# Autodesk Inventor assembly: emsamble caja
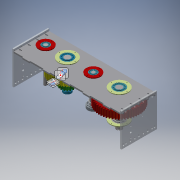
[picture p0: Inventor's stored thumbnail of the model, 180x180]
Saved by Autodesk Inventor 2016 (Build 200138000, 138)
## iProperties
Created: 2017-08-31
Part Number: emsamble caja
Material: Genérico
Document SubType Name: Assembly
Designer: Alumno
Author: Alumno
## Documents named in this file (20)
- C:\Users\Alumno\Desktop\proyecto caja reductora\emsamble caja.iam
- C:\Users\Alumno\Desktop\proyecto caja reductora\Acople N°1.ipt
- C:\Users\Alumno\Desktop\proyecto caja reductora\Plano 2.ipt
- C:\Users\Alumno\Desktop\proyecto caja reductora\AcoplecN°2.ipt
- C:\Users\Alumno\Desktop\proyecto caja reductora\EJE 2 (30 mm y 15 mm).iam
- C:\Users\Alumno\Desktop\proyecto caja reductora\TREN 1\Design Accelerator\Engranaje recto12.ipt
- C:\Users\Alumno\Desktop\proyecto caja reductora\TREN 1\Design Accelerator\Engranaje recto22.ipt
- C:\Users\Alumno\Desktop\proyecto caja reductora\TREN 2\Design Accelerator\Engranaje recto11.ipt
- C:\Users\Alumno\Desktop\proyecto caja reductora\TREN 2\Design Accelerator\Engranaje recto21.ipt
- C:\Users\Alumno\Desktop\proyecto caja reductora\TREN 3\Design Accelerator\Engranaje recto11.ipt
- C:\Users\Alumno\Desktop\proyecto caja reductora\TREN 3\Design Accelerator\Engranaje recto21.ipt
- C:\Users\Alumno\Desktop\proyecto caja reductora\EJE 3 (30-45).iam
- C:\Users\Alumno\Desktop\proyecto caja reductora\EJE 4.iam
- C:\Users\Alumno\Desktop\proyecto caja reductora\Chaveta- Tren 1.ipt
- C:\Users\Alumno\Desktop\proyecto caja reductora\Chaveta 25.ipt
- C:\Users\Alumno\Desktop\proyecto caja reductora\EJE 1.iam
- C:\Users\Alumno\Desktop\proyecto caja reductora\RODAMIENTO 15 D\6002.iam
- C:\Users\Alumno\Desktop\proyecto caja reductora\RODAMIENTO 25 D\6005.iam
- C:\Users\Alumno\Desktop\proyecto caja reductora\PLANO  N°1.ipt
- C:\Users\Alumno\Desktop\proyecto caja reductora\PLANO N°2.ipt
## Components (33 placed, 15 different names)
1. Engranaje recto1:1 — Rotación:4, Coincidencia:138, Coincidencia:139, Coincidencia:184
2. Engranaje recto2:1 — Coincidencia:120, Coincidencia:121, Coincidencia:132, Rotación:4
3. Engranaje recto2:2 — Coincidencia:212, Coincidencia:213, Coincidencia:214, Rotación:7
4. Engranaje recto1:3 — Coincidencia:99, Coincidencia:114, Coincidencia:135, Rotación:6
5. Engranaje recto2:3 — Coincidencia:112, Coincidencia:125, Rotación:6, Coincidencia:206
6. EJE 2 (30 mm y 15 mm):3 [sub-assembly] — Coincidencia:94, Coincidencia:95, Coincidencia:117, Coincidencia:118, Coincidencia:119, Coincidencia:120, Coincidencia:132, Coincidencia:134, Coincidencia:202, Nivelación:5, Coincidencia:230
7. Engranaje recto1:4 — Coincidencia:94, Coincidencia:95, Coincidencia:134, Rotación:7
8. EJE 3 (30-45):1 [sub-assembly] — Coincidencia:99, Coincidencia:114, Coincidencia:127, Coincidencia:128, Coincidencia:129, Coincidencia:135, Coincidencia:203, Nivelación:6, Coincidencia:205, Coincidencia:213, Coincidencia:214
9. EJE 4:1 [sub-assembly] — Coincidencia:112, Coincidencia:122, Coincidencia:123, Coincidencia:124, Coincidencia:204, Nivelación:7, Coincidencia:206
10. Chaveta- Tren 1:1 — Coincidencia:117, Coincidencia:118, Coincidencia:119, Coincidencia:121
11. Chaveta- Tren 1:2 — Coincidencia:122, Coincidencia:123, Coincidencia:124, Coincidencia:125
12. Chaveta 25:6 — Coincidencia:127, Coincidencia:128, Coincidencia:129, Coincidencia:205, Coincidencia:212
13. EJE 1:1 [sub-assembly] — Coincidencia:138, Coincidencia:139, Coincidencia:169, Coincidencia:184, Coincidencia:201, Nivelación:4, Coincidencia:229
14. 6002:3 [sub-assembly] — Coincidencia:169, Coincidencia:197, Nivelación:1, Coincidencia:201, Nivelación:4
15. 6002:4 [sub-assembly] — Coincidencia:199, Nivelación:2, Coincidencia:203, Nivelación:6
16. 6005:3 [sub-assembly] — Coincidencia:200, Nivelación:3, Coincidencia:204, Nivelación:7
17. PLANO  N°1:1 — Coincidencia:185, Coincidencia:186, Coincidencia:187, Coincidencia:188, Coincidencia:189, Coincidencia:190, Coincidencia:191, Coincidencia:192, Coincidencia:193, Coincidencia:194, Coincidencia:195, Coincidencia:196, Nivelación:9, Coincidencia:208, Coincidencia:209, Coincidencia:233, Nivelación:15, Coincidencia:234
18. Acople N°1:2 — Coincidencia:186, Coincidencia:188, Coincidencia:189, Coincidencia:197, Nivelación:1
19. Acople N°1:3 — Coincidencia:185, Coincidencia:187, Coincidencia:190, Coincidencia:199, Nivelación:2
20. AcoplecN°2:1 — Coincidencia:191, Coincidencia:194, Coincidencia:196, Coincidencia:198, Nivelación:8
21. AcoplecN°2:2 — Coincidencia:192, Coincidencia:193, Coincidencia:195, Coincidencia:200, Nivelación:3
22. 6005:5 [sub-assembly] — Coincidencia:198, Coincidencia:202, Nivelación:5, Nivelación:8
23. Plano 2:1 — Nivelación:9, Coincidencia:208, Coincidencia:209, Nivelación:10, Coincidencia:215, Coincidencia:216
24. PLANO N°2:1 — Nivelación:10, Coincidencia:215, Coincidencia:216, Coincidencia:217, Coincidencia:218, Coincidencia:219, Coincidencia:220, Coincidencia:221, Coincidencia:222, Coincidencia:223, Coincidencia:224, Coincidencia:225, Coincidencia:226, Coincidencia:227, Coincidencia:228
25. AcoplecN°2:3 — Coincidencia:218, Coincidencia:222, Coincidencia:226, Coincidencia:231, Nivelación:13
26. Acople N°1:4 — Coincidencia:219, Coincidencia:223, Coincidencia:228, Nivelación:12
27. AcoplecN°2:4 — Coincidencia:217, Coincidencia:221, Coincidencia:227, Coincidencia:232, Nivelación:14
28. Acople N°1:5 — Coincidencia:220, Coincidencia:224, Coincidencia:225, Nivelación:11
29. 6002:5 [sub-assembly] — Coincidencia:229, Nivelación:11
30. 6002:6 [sub-assembly] — Coincidencia:230, Nivelación:12
31. 6005:6 [sub-assembly] — Coincidencia:231, Nivelación:13
32. 6005:7 [sub-assembly] — Coincidencia:232, Nivelación:14
33. Plano 2:2 — Coincidencia:233, Nivelación:15, Coincidencia:234
## Relationships (89: Mate 71, Flush 15, RelateRotation 3)
- Coincidencia:94 [Mate]: EJE 2 (30 mm y 15 mm):3 ↔ Engranaje recto1:4
- Coincidencia:95 [Mate]: EJE 2 (30 mm y 15 mm):3 ↔ Engranaje recto1:4
- Coincidencia:99 [Mate]: Engranaje recto1:3 ↔ EJE 3 (30-45):1
- Coincidencia:112 [Mate]: Engranaje recto2:3 ↔ EJE 4:1
- Coincidencia:114 [Mate]: Engranaje recto1:3 ↔ EJE 3 (30-45):1
- Coincidencia:117 [Mate]: EJE 2 (30 mm y 15 mm):3 ↔ Chaveta- Tren 1:1
- Coincidencia:118 [Mate]: EJE 2 (30 mm y 15 mm):3 ↔ Chaveta- Tren 1:1
- Coincidencia:119 [Mate]: EJE 2 (30 mm y 15 mm):3 ↔ Chaveta- Tren 1:1
- Coincidencia:120 [Mate]: Engranaje recto2:1 ↔ EJE 2 (30 mm y 15 mm):3
- Coincidencia:121 [Mate]: Engranaje recto2:1 ↔ Chaveta- Tren 1:1
- Coincidencia:122 [Mate]: EJE 4:1 ↔ Chaveta- Tren 1:2
- Coincidencia:123 [Mate]: EJE 4:1 ↔ Chaveta- Tren 1:2
- Coincidencia:124 [Mate]: EJE 4:1 ↔ Chaveta- Tren 1:2
- Coincidencia:125 [Mate]: Engranaje recto2:3 ↔ Chaveta- Tren 1:2
- Coincidencia:127 [Mate]: EJE 3 (30-45):1 ↔ Chaveta 25:6
- Coincidencia:128 [Mate]: EJE 3 (30-45):1 ↔ Chaveta 25:6
- Coincidencia:129 [Mate]: EJE 3 (30-45):1 ↔ Chaveta 25:6
- Coincidencia:132 [Mate]: Engranaje recto2:1 ↔ EJE 2 (30 mm y 15 mm):3
- Coincidencia:134 [Mate]: EJE 2 (30 mm y 15 mm):3 ↔ Engranaje recto1:4
- Coincidencia:135 [Mate]: Engranaje recto1:3 ↔ EJE 3 (30-45):1
- Rotación:4 [RelateRotation] (0.3333 ul): Engranaje recto1:1 ↔ Engranaje recto2:1
- Rotación:6 [RelateRotation] (0.3333 ul): Engranaje recto1:3 ↔ Engranaje recto2:3
- Coincidencia:138 [Mate]: Engranaje recto1:1 ↔ EJE 1:1
- Coincidencia:139 [Mate]: Engranaje recto1:1 ↔ EJE 1:1
- Coincidencia:169 [Mate]: EJE 1:1 ↔ 6002:3
- Coincidencia:184 [Mate]: Engranaje recto1:1 ↔ EJE 1:1
- Coincidencia:185 [Mate]: PLANO  N°1:1 ↔ Acople N°1:3
- Coincidencia:186 [Mate]: PLANO  N°1:1 ↔ Acople N°1:2
- Coincidencia:187 [Mate]: PLANO  N°1:1 ↔ Acople N°1:3
- Coincidencia:188 [Mate]: PLANO  N°1:1 ↔ Acople N°1:2
- Coincidencia:189 [Mate]: PLANO  N°1:1 ↔ Acople N°1:2
- Coincidencia:190 [Mate]: PLANO  N°1:1 ↔ Acople N°1:3
- Coincidencia:191 [Mate]: PLANO  N°1:1 ↔ AcoplecN°2:1
- Coincidencia:192 [Mate]: PLANO  N°1:1 ↔ AcoplecN°2:2
- Coincidencia:193 [Mate]: PLANO  N°1:1 ↔ AcoplecN°2:2
- Coincidencia:194 [Mate]: PLANO  N°1:1 ↔ AcoplecN°2:1
- Coincidencia:195 [Mate]: PLANO  N°1:1 ↔ AcoplecN°2:2
- Coincidencia:196 [Mate]: PLANO  N°1:1 ↔ AcoplecN°2:1
- Coincidencia:197 [Mate]: 6002:3 ↔ Acople N°1:2
- Nivelación:1 [Flush]: 6002:3 ↔ Acople N°1:2
- Coincidencia:198 [Mate]: AcoplecN°2:1 ↔ 6005:5
- Coincidencia:199 [Mate]: 6002:4 ↔ Acople N°1:3
- Nivelación:2 [Flush]: 6002:4 ↔ Acople N°1:3
- Coincidencia:200 [Mate]: 6005:3 ↔ AcoplecN°2:2
- Nivelación:3 [Flush]: 6005:3 ↔ AcoplecN°2:2
- Coincidencia:201 [Mate]: EJE 1:1 ↔ 6002:3
- Nivelación:4 [Flush]: EJE 1:1 ↔ 6002:3
- Coincidencia:202 [Mate]: EJE 2 (30 mm y 15 mm):3 ↔ 6005:5
- Nivelación:5 [Flush]: EJE 2 (30 mm y 15 mm):3 ↔ 6005:5
- Coincidencia:203 [Mate]: EJE 3 (30-45):1 ↔ 6002:4
- Nivelación:6 [Flush]: EJE 3 (30-45):1 ↔ 6002:4
- Coincidencia:204 [Mate]: EJE 4:1 ↔ 6005:3
- Nivelación:7 [Flush]: EJE 4:1 ↔ 6005:3
- Coincidencia:205 [Mate]: EJE 3 (30-45):1 ↔ Chaveta 25:6
- Coincidencia:206 [Mate]: Engranaje recto2:3 ↔ EJE 4:1
- Nivelación:8 [Flush]: AcoplecN°2:1 ↔ 6005:5
- Nivelación:9 [Flush]: PLANO  N°1:1 ↔ Plano 2:1
- Coincidencia:208 [Mate]: PLANO  N°1:1 ↔ Plano 2:1
- Coincidencia:209 [Mate]: PLANO  N°1:1 ↔ Plano 2:1
- Coincidencia:212 [Mate]: Engranaje recto2:2 ↔ Chaveta 25:6
- Coincidencia:213 [Mate]: Engranaje recto2:2 ↔ EJE 3 (30-45):1
- Coincidencia:214 [Mate]: Engranaje recto2:2 ↔ EJE 3 (30-45):1
- Rotación:7 [RelateRotation] (0.3333 ul): Engranaje recto2:2 ↔ Engranaje recto1:4
- Nivelación:10 [Flush]: Plano 2:1 ↔ PLANO N°2:1
- Coincidencia:215 [Mate]: Plano 2:1 ↔ PLANO N°2:1
- Coincidencia:216 [Mate]: Plano 2:1 ↔ PLANO N°2:1
- Coincidencia:217 [Mate]: PLANO N°2:1 ↔ AcoplecN°2:4
- Coincidencia:218 [Mate]: PLANO N°2:1 ↔ AcoplecN°2:3
- Coincidencia:219 [Mate]: PLANO N°2:1 ↔ Acople N°1:4
- Coincidencia:220 [Mate]: PLANO N°2:1 ↔ Acople N°1:5
- Coincidencia:221 [Mate]: PLANO N°2:1 ↔ AcoplecN°2:4
- Coincidencia:222 [Mate]: PLANO N°2:1 ↔ AcoplecN°2:3
- Coincidencia:223 [Mate]: PLANO N°2:1 ↔ Acople N°1:4
- Coincidencia:224 [Mate]: PLANO N°2:1 ↔ Acople N°1:5
- Coincidencia:225 [Mate]: PLANO N°2:1 ↔ Acople N°1:5
- Coincidencia:226 [Mate]: PLANO N°2:1 ↔ AcoplecN°2:3
- Coincidencia:227 [Mate]: PLANO N°2:1 ↔ AcoplecN°2:4
- Coincidencia:228 [Mate]: PLANO N°2:1 ↔ Acople N°1:4
- Coincidencia:229 [Mate]: EJE 1:1 ↔ 6002:5
- Nivelación:11 [Flush]: Acople N°1:5 ↔ 6002:5
- Coincidencia:230 [Mate]: EJE 2 (30 mm y 15 mm):3 ↔ 6002:6
- Nivelación:12 [Flush]: Acople N°1:4 ↔ 6002:6
- Coincidencia:231 [Mate]: AcoplecN°2:3 ↔ 6005:6
- Nivelación:13 [Flush]: AcoplecN°2:3 ↔ 6005:6
- Coincidencia:232 [Mate]: AcoplecN°2:4 ↔ 6005:7
- Nivelación:14 [Flush]: AcoplecN°2:4 ↔ 6005:7
- Coincidencia:233 [Mate]: PLANO  N°1:1 ↔ Plano 2:2
- Nivelación:15 [Flush]: PLANO  N°1:1 ↔ Plano 2:2
- Coincidencia:234 [Mate]: PLANO  N°1:1 ↔ Plano 2:2
